# Autodesk Inventor assembly: A02 - Main Shaft Assembly
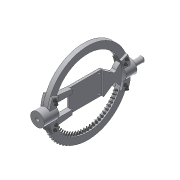
[picture p0: Inventor's stored thumbnail of the model, 180x180]
Saved by Autodesk Inventor 2016 (Build 200138000, 138)
## iProperties
Created: 2016-12-26
Part Number: A02 - Main Shaft Assembly
Document SubType Name: Conjunto soldado
Designer: Fernando
Weld Material: Aço macio soldado
Mass: 165.083 g
Surface Area: 719.908 cm^2
Volume: 155.862 cm^3
Density: 1.05916 g/cm^3
SurfaceArea_m2: .07
Author: Fernando
## Documents named in this file (7)
- G:\00 - Files\00 - Personal\40 - Hobbies\90 - Projetos Particulares\40 - POV Display\01 - Mechanical Design\A02 - Main Shaft Assembly.iam
- G:\00 - Files\00 - Personal\40 - Hobbies\90 - Projetos Particulares\40 - POV Display\01 - Mechanical Design\M03 - Shaft Component 1.ipt
- G:\00 - Files\00 - Personal\40 - Hobbies\90 - Projetos Particulares\40 - POV Display\01 - Mechanical Design\M02 - Main Spherical Shaft.ipt
- G:\00 - Files\00 - Personal\40 - Hobbies\90 - Projetos Particulares\40 - POV Display\01 - Mechanical Design\M04 - Shaft Component 2.ipt
- G:\00 - Files\00 - Personal\40 - Hobbies\90 - Projetos Particulares\40 - POV Display\01 - Mechanical Design\P02 - LED 5mm.ipt
- G:\00 - Files\00 - Personal\40 - Hobbies\90 - Projetos Particulares\40 - POV Display\01 - Mechanical Design\P06 - M3 Bolt.ipt
- G:\00 - Files\00 - Personal\40 - Hobbies\90 - Projetos Particulares\40 - POV Display\01 - Mechanical Design\P05 - M3 Nut.ipt
## Components (45 placed, 6 different names)
1. M03 - Shaft Component 1:2 — Mate:1, Mate:2, Mate:3, Insert:2, Insert:3, Insert:4, Insert:5, Insert:10, Insert:11, Insert:16, Insert:17
2. M02 - Main Spherical Shaft:1 — Mate:1, Mate:2, Mate:3, Mate:4, Mate:5, Mate:6, Insert:1
3. M04 - Shaft Component 2:1 — Mate:4, Mate:5, Mate:6, Insert:6, Insert:7, Insert:8, Insert:9, Insert:12, Insert:13, Insert:14, Insert:15
4. P06 - M3 Bolt:1 — Insert:2
5. P05 - M3 Nut:1 — Insert:5
6. P06 - M3 Bolt:2 — Insert:3
7. P05 - M3 Nut:2 — Insert:4
8. P06 - M3 Bolt:3 — Insert:17
9. P05 - M3 Nut:3 — Insert:11
10. P06 - M3 Bolt:4 — Insert:16
11. P05 - M3 Nut:4 — Insert:10
12. P06 - M3 Bolt:5 — Insert:12
13. P05 - M3 Nut:5 — Insert:7
14. P06 - M3 Bolt:6 — Insert:13
15. P05 - M3 Nut:6 — Insert:6
16. P06 - M3 Bolt:7 — Insert:15
17. P05 - M3 Nut:7 — Insert:9
18. P06 - M3 Bolt:8 — Insert:14
19. P05 - M3 Nut:8 — Insert:8
20. P02 - LED 5mm:1 — Insert:1
21. P02 - LED 5mm:2
22. P02 - LED 5mm:3
23. P02 - LED 5mm:4
24. P02 - LED 5mm:5
25. P02 - LED 5mm:6
26. P02 - LED 5mm:7
27. P02 - LED 5mm:8
28. P02 - LED 5mm:9
29. P02 - LED 5mm:10
30. P02 - LED 5mm:11
31. P02 - LED 5mm:12
32. P02 - LED 5mm:13
33. P02 - LED 5mm:14
34. P02 - LED 5mm:15
35. P02 - LED 5mm:16
36. P02 - LED 5mm:17
37. P02 - LED 5mm:18
38. P02 - LED 5mm:19
39. P02 - LED 5mm:20
40. P02 - LED 5mm:21
41. P02 - LED 5mm:22
42. P02 - LED 5mm:23
43. P02 - LED 5mm:24
44. P02 - LED 5mm:25
45. P02 - LED 5mm:26
## Component patterns: (26 elements, first: P02 - LED 5mm:1)
## Relationships (23: Insert 17, Mate 6)
- Mate:1: M03 - Shaft Component 1:2 ↔ M02 - Main Spherical Shaft:1
- Mate:2: M03 - Shaft Component 1:2 ↔ M02 - Main Spherical Shaft:1
- Mate:3: M03 - Shaft Component 1:2 ↔ M02 - Main Spherical Shaft:1
- Mate:4: M02 - Main Spherical Shaft:1 ↔ M04 - Shaft Component 2:1
- Mate:5: M02 - Main Spherical Shaft:1 ↔ M04 - Shaft Component 2:1
- Mate:6: M02 - Main Spherical Shaft:1 ↔ M04 - Shaft Component 2:1
- Insert:1: M02 - Main Spherical Shaft:1 ↔ P02 - LED 5mm:1
- Insert:2: M03 - Shaft Component 1:2 ↔ P06 - M3 Bolt:1
- Insert:3: M03 - Shaft Component 1:2 ↔ P06 - M3 Bolt:2
- Insert:4: M03 - Shaft Component 1:2 ↔ P05 - M3 Nut:2
- Insert:5: M03 - Shaft Component 1:2 ↔ P05 - M3 Nut:1
- Insert:6: M04 - Shaft Component 2:1 ↔ P05 - M3 Nut:6
- Insert:7: M04 - Shaft Component 2:1 ↔ P05 - M3 Nut:5
- Insert:8: M04 - Shaft Component 2:1 ↔ P05 - M3 Nut:8
- Insert:9: M04 - Shaft Component 2:1 ↔ P05 - M3 Nut:7
- Insert:10: M03 - Shaft Component 1:2 ↔ P05 - M3 Nut:4
- Insert:11: M03 - Shaft Component 1:2 ↔ P05 - M3 Nut:3
- Insert:12: M04 - Shaft Component 2:1 ↔ P06 - M3 Bolt:5
- Insert:13: M04 - Shaft Component 2:1 ↔ P06 - M3 Bolt:6
- Insert:14: M04 - Shaft Component 2:1 ↔ P06 - M3 Bolt:8
- Insert:15: M04 - Shaft Component 2:1 ↔ P06 - M3 Bolt:7
- Insert:16: M03 - Shaft Component 1:2 ↔ P06 - M3 Bolt:4
- Insert:17: M03 - Shaft Component 1:2 ↔ P06 - M3 Bolt:3
